# Autodesk Inventor assembly: Chamber_assembly
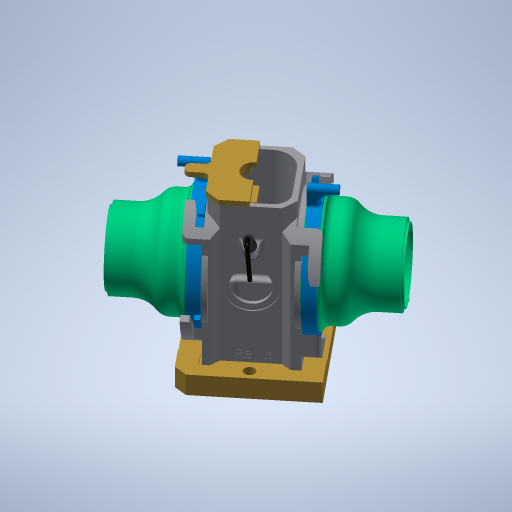
[picture p0: Inventor's stored thumbnail of the model, 512x512]
Saved by Autodesk Inventor 2023.3 (Build 273359000, 359)
## iProperties
Created: 2023-03-24
Part Number: Chamber_assembly
Document SubType Name: Assembly
Designer: ak-stelzer
Author: ak-stelzer
## Documents named in this file (7)
- C:\Users\ak-stelzer\source\repos\artgolden\light_sheet_specimen_chambers\Flexible seal for high NA objectives\Specimen_chamber_example\Chamber_assembly.iam
- C:\Users\ak-stelzer\source\repos\artgolden\light_sheet_specimen_chambers\Flexible seal for high NA objectives\Specimen_chamber_example\Sealing_ring_20x1_silicone_i.ipt
- C:\Users\ak-stelzer\source\repos\artgolden\light_sheet_specimen_chambers\Flexible seal for high NA objectives\Specimen_chamber_example\Sealing_silicone_h.ipt
- C:\Users\ak-stelzer\source\repos\artgolden\light_sheet_specimen_chambers\Flexible seal for high NA objectives\Specimen_chamber_example\Chamber_lid.ipt
- C:\Users\ak-stelzer\source\repos\artgolden\light_sheet_specimen_chambers\Flexible seal for high NA objectives\Specimen_chamber_example\TempSensor_RS-762-1134.ipt
- C:\Users\ak-stelzer\source\repos\artgolden\light_sheet_specimen_chambers\Flexible seal for high NA objectives\Specimen_chamber_example\dsDSLM_Chamber_2.0_k.ipt
- C:\Users\ak-stelzer\source\repos\artgolden\light_sheet_specimen_chambers\Flexible seal for high NA objectives\Specimen_chamber_example\ChamberMount_c.ipt
## Components (8 placed, 6 different names)
1. dsDSLM_Chamber_2.0_k:1
2. Sealing_ring_20x1_silicone_i:3
3. Sealing_silicone_h:3
4. ChamberMount_c:2
5. Chamber_lid:1
6. Sealing_ring_20x1_silicone_i:2
7. Sealing_silicone_h:2
8. TempSensor_RS-762-1134:2
## Relationships (13: Mate 8, RevoluteJoint 5)
- [Mate]: dsDSLM_Chamber_2.0_k:1
- [Mate]: dsDSLM_Chamber_2.0_k:1 ↔ ChamberMount_c:2
- [Mate]: dsDSLM_Chamber_2.0_k:1 ↔ ChamberMount_c:2
- [Mate]: dsDSLM_Chamber_2.0_k:1 ↔ ChamberMount_c:2
- [RevoluteJoint]: Sealing_ring_20x1_silicone_i:3 ↔ Sealing_silicone_h:3
- [RevoluteJoint]: dsDSLM_Chamber_2.0_k:1 ↔ Sealing_ring_20x1_silicone_i:3
- [Mate]: Sealing_ring_20x1_silicone_i:3 ↔ Sealing_silicone_h:3
- [RevoluteJoint]: Sealing_ring_20x1_silicone_i:2 ↔ Sealing_silicone_h:2
- [Mate]: Sealing_ring_20x1_silicone_i:2 ↔ Sealing_silicone_h:2
- [RevoluteJoint]: dsDSLM_Chamber_2.0_k:1 ↔ Sealing_silicone_h:2
- [Mate]: dsDSLM_Chamber_2.0_k:1 ↔ Chamber_lid:1
- [Mate]: dsDSLM_Chamber_2.0_k:1 ↔ Chamber_lid:1
- [RevoluteJoint]: dsDSLM_Chamber_2.0_k:1 ↔ TempSensor_RS-762-1134:2
## Named parameters: d11_d4 = 0 mm, d12_d5 = 123 deg, d13_d10 = 0 mm
